# Autodesk Inventor assembly: Confirmat Joint13
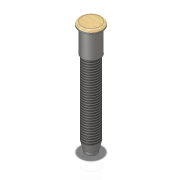
[picture p0: Inventor's stored thumbnail of the model, 180x180]
Saved by Autodesk Inventor 2024 (Build 280153000, 153)
## iProperties
RuleStatus: InUse
AfterAnyUserParamChange0: Pass Partameters
Created: 2023-01-24
Part Number: Confirmat Joint13
Document SubType Name: Assembly
Designer: sauliusd
Author: sauliusd
## Documents named in this file (3)
- C:\W4INV 2024 Design\PROJECTS\Samples\Macro DEMO\7 Computer Case\Computer Case.iam Smart Hardware\Confirmat Joint13\Confirmat Joint13.iam
- C:\W4INV 2024 Design\PROJECTS\Samples\Macro DEMO\7 Computer Case\Computer Case.iam Smart Hardware\Confirmat Joint13\Confirmat Joint1300.ipt
- C:\W4INV 2024 Design\PROJECTS\Samples\Macro DEMO\7 Computer Case\Computer Case.iam Smart Hardware\Confirmat Joint13\Confirmat Joint1301.iam
## Components (3 placed, 3 different names)
1. @Skeleton — Flush:1, Flush:2, Flush:3, Insert:1
2. Confirmat&Cap [sub-assembly] — Insert:1
3. Confirmat Joint1301:2 [sub-assembly]
## Component patterns: (2 elements, first: Confirmat&Cap)
## Relationships (4: Flush 3, Insert 1)
- Flush:1: @Skeleton
- Flush:2: @Skeleton
- Flush:3: @Skeleton
- Insert:1: @Skeleton ↔ Confirmat&Cap
## Named parameters: ContactPatchWidth = 264 mm, ContactPatchHeight = 18 mm, NesteledBoardThickness = 18 mm, Gap = 0 mm, ConnectionAngle = 90 deg, MaxAllowedDistance = 300 mm, ShiftFromSide1 = 60 mm, ShiftFromSide2 = 60 mm, MinAllowedDistance = 20 mm
